# Autodesk Inventor assembly: hood
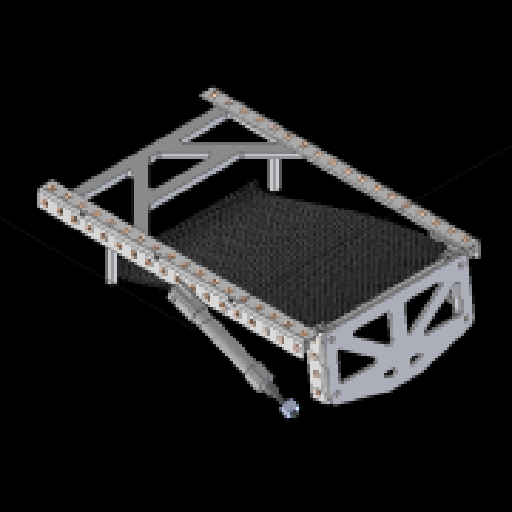
[picture p0: Inventor's stored thumbnail of the model, 512x512]
Saved by Autodesk Inventor 2025.2 (Build 292293000, 293)
## iProperties
Created: 2025-12-05
Part Number: hood
Document SubType Name: Assembly
Designer: cloudy
Author: cloudy
## Documents named in this file (15)
- C:\Users\cloudy\Documents\AURA_CAD\15\hood.iam
- C:\Users\cloudy\Documents\AURA_CAD\!lib\Structure\C Channel\Aluminum 1x3x1 Half\Alu C Half 1x3x1x18.ipt
- C:\Users\cloudy\Documents\AURA_CAD\15\hoodbrace.ipt
- C:\Users\cloudy\Documents\AURA_CAD\15\25 stroke 10 bore\CJ2D10-25Z(0_0).iam
- C:\Users\cloudy\Documents\AURA_CAD\!lib\Structure\C Channel\Aluminum 1x3x1 Half\Alu C Half 1x3x1x4.ipt
- C:\Users\cloudy\Documents\AURA_CAD\!lib\Motion\Shaft LS\Shaft Collar Metal\Shaft Collar No Screw.iam
- C:\Users\cloudy\Documents\GitHub\aura-cad\!lib\Motion\Shaft LS\Shaft Collar Metal.iam
- C:\Users\cloudy\Documents\AURA_CAD\15\rangoon.ipt
- C:\Users\cloudy\Documents\AURA_CAD\!lib\Structure\Standoff\Standoff 4.00.ipt
- C:\Users\cloudy\Documents\GitHub\aura-cad\!lib\Structure\Standoff.ipt
- C:\Users\cloudy\Documents\AURA_CAD\!lib\Motion\Spacers\Spacer Nylon .375 OD\NSpacer .375 OD x .125.ipt
- C:\Users\cloudy\Documents\GitHub\aura-cad\!lib\Motion\Spacers\Spacer Nylon .375 OD.ipt
- C:\Users\cloudy\Documents\AURA_CAD\!lib\Motion\Shaft LS\Bearing Flat.ipt
- C:\Users\cloudy\Documents\AURA_CAD\!lib\Structure\Standoff\Standoff 1.50.ipt
- C:\Users\cloudy\Documents\AURA_CAD\15\mesh.ipt
## Components (18 placed, 11 different names)
1. Alu C Half 1x3x1x18:1 — Insert:1, Mate:1, Insert:7, Insert:10, Mate:7
2. Alu C Half 1x3x1x18:2 — Insert:1, Mate:1, Flush:1, Mate:3, Insert:5, Insert:9, Mate:6
3. hoodbrace:1 — Flush:1, Insert:16, Insert:17
4. CJ2D10-25Z(0_0):1 [sub-assembly] — Mate:3, Insert:4
5. Alu C Half 1x3x1x4:2 — Insert:7, Mate:4, Insert:15, Mate:9
6. Shaft Collar No Screw:1 [sub-assembly] — Insert:4, Insert:6
7. Alu C Half 1x3x1x4:3 — Insert:5, Insert:6, Mate:4, Flush:2, Insert:8, Mate:5, Flush:3
8. rangoon:1 — Flush:2, Insert:8, Mate:5
9. Standoff 4.00:1 — Insert:11, Insert:12
10. NSpacer .375 OD x .125:1 — Insert:12, Insert:13
11. NSpacer .375 OD x .125:2 — Insert:11, Insert:14
12. Bearing Flat:1 — Insert:10, Mate:7
13. Bearing Flat:2 — Insert:9, Mate:6
14. Bearing Flat:3 — Insert:14, Mate:8
15. Bearing Flat:4 — Insert:13, Mate:8, Insert:15, Mate:9
16. Standoff 1.50:2 — Insert:16
17. Standoff 1.50:3 — Insert:17
18. mesh:1 — Flush:3
## Relationships (26: Insert 15, Mate 8, Flush 3)
- Insert:1 (-152.4 mm): Alu C Half 1x3x1x18:1 ↔ Alu C Half 1x3x1x18:2
- Mate:1: Alu C Half 1x3x1x18:1 ↔ Alu C Half 1x3x1x18:2
- Flush:1: Alu C Half 1x3x1x18:2 ↔ hoodbrace:1
- Mate:3: Alu C Half 1x3x1x18:2 ↔ CJ2D10-25Z(0_0):1
- Insert:4 (3 mm): CJ2D10-25Z(0_0):1 ↔ Shaft Collar No Screw:1
- Insert:5 (12.7 mm): Alu C Half 1x3x1x18:2 ↔ Alu C Half 1x3x1x4:3
- Insert:6 (19.05 mm): Shaft Collar No Screw:1 ↔ Alu C Half 1x3x1x4:3
- Insert:7 (12.7 mm): Alu C Half 1x3x1x18:1 ↔ Alu C Half 1x3x1x4:2
- Mate:4: Alu C Half 1x3x1x4:2 ↔ Alu C Half 1x3x1x4:3
- Flush:2: Alu C Half 1x3x1x4:3 ↔ rangoon:1
- Insert:8: Alu C Half 1x3x1x4:3 ↔ rangoon:1
- Mate:5: Alu C Half 1x3x1x4:3 ↔ rangoon:1
- Insert:9: Alu C Half 1x3x1x18:2 ↔ Bearing Flat:2
- Mate:6: Alu C Half 1x3x1x18:2 ↔ Bearing Flat:2
- Insert:10: Alu C Half 1x3x1x18:1 ↔ Bearing Flat:1
- Mate:7: Alu C Half 1x3x1x18:1 ↔ Bearing Flat:1
- Insert:11: Standoff 4.00:1 ↔ NSpacer .375 OD x .125:2
- Insert:12: Standoff 4.00:1 ↔ NSpacer .375 OD x .125:1
- Insert:13: NSpacer .375 OD x .125:1 ↔ Bearing Flat:4
- Insert:14: NSpacer .375 OD x .125:2 ↔ Bearing Flat:3
- Mate:8: Bearing Flat:3 ↔ Bearing Flat:4
- Insert:15: Alu C Half 1x3x1x4:2 ↔ Bearing Flat:4
- Mate:9: Alu C Half 1x3x1x4:2 ↔ Bearing Flat:4
- Insert:16: hoodbrace:1 ↔ Standoff 1.50:2
- Insert:17: hoodbrace:1 ↔ Standoff 1.50:3
- Flush:3: Alu C Half 1x3x1x4:3 ↔ mesh:1
